# Autodesk Inventor assembly: Assembly1
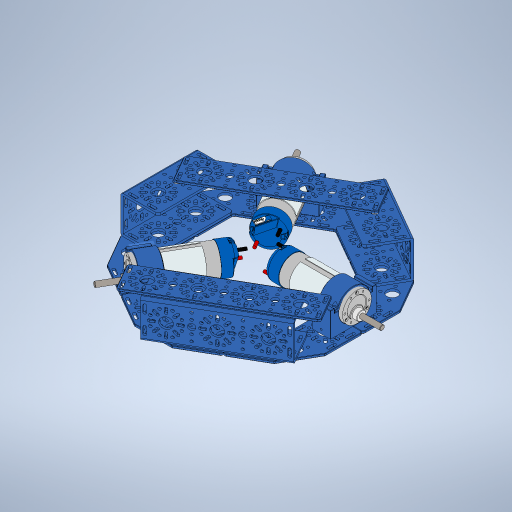
[picture p0: Inventor's stored thumbnail of the model, 512x512]
Saved by Autodesk Inventor 2023 (Build 270158000, 158)
## iProperties
Created: 2022-11-05
Part Number: Assembly1
Document SubType Name: Assembly
Designer: amagw
Author: amagw
## Documents named in this file (9)
- C:\Users\amagw\OneDrive\Документы\Inventor\Assembly1.iam
- C:\Users\amagw\Downloads\76080-120-degree-bracket.ipt
- C:\Users\amagw\Downloads\76017-96mm-u-channel.ipt
- C:\Users\amagw\Downloads\76016-144mm-u-channel.ipt
- C:\Users\amagw\Downloads\76141b-motor-mount-clamp-bottom.ipt
- C:\Users\amagw\Downloads\75001 - Maverick Motor, Spur Gearbox and Encoder.ipt
- C:\Users\amagw\Downloads\76141t-motor-mount-clamp-kit-top.ipt
- C:\Users\amagw\Downloads\76063-192mm-40mm-flat-bracket(1).ipt
- C:\Users\amagw\Downloads\76063-192mm-40mm-flat-bracket(2).ipt
## Components (20 placed, 8 different names)
1. 76063-192mm-40mm-flat-bracket(1):1 — Angle:7, Rotational:14, Rotational:15
2. 76063-192mm-40mm-flat-bracket(2):1 — Angle:8, Rotational:17
3. 76017-96mm-u-channel:2 — Rotational:1, Rotational:2
4. 76016-144mm-u-channel:2 — Rotational:6, Rotational:7, Angle:7, Rotational:14, Rotational:15
5. 76017-96mm-u-channel:1 — Rotational:3, Rotational:4, Rotational:17
6. 76080-120-degree-bracket:1 — Rigid:1, Rotational:6, Rotational:7
7. 76080-120-degree-bracket:2 — Rigid:1, Rigid:2, Rotational:8, Angle:1, Angle:6
8. 76080-120-degree-bracket:3 — Rigid:2, Rigid:3, Rotational:1
9. 76080-120-degree-bracket:4 — Rigid:3, Rigid:4, Rotational:2, Angle:3, Angle:8
10. 76080-120-degree-bracket:5 — Rigid:4, Rigid:5, Rotational:3, Angle:2
11. 76080-120-degree-bracket:6 — Rigid:5, Rotational:4, Angle:4, Angle:5
12. 76141b-motor-mount-clamp-bottom:1 — Angle:4, Angle:5, Rigid:6, Rotational:13, Rotational:16
13. 76141b-motor-mount-clamp-bottom:2 — Angle:2, Angle:3, Rigid:9, Rotational:9, Rotational:10
14. 76141b-motor-mount-clamp-bottom:3 — Rotational:8, Angle:1, Angle:6, Rigid:8, Rotational:11, Rotational:12
15. 75001 - Maverick Motor, Spur Gearbox and Encoder:1 — Rigid:6
16. 75001 - Maverick Motor, Spur Gearbox and Encoder:2 — Rigid:8
17. 75001 - Maverick Motor, Spur Gearbox and Encoder:3 — Rigid:9
18. 76141t-motor-mount-clamp-kit-top:1 — Rotational:11, Rotational:12
19. 76141t-motor-mount-clamp-kit-top:2 — Rotational:13, Rotational:16
20. 76141t-motor-mount-clamp-kit-top:3 — Rotational:9, Rotational:10
## Relationships (32: RevoluteJoint 16, WeldJoint 8, Angle 8)
- Rigid:1 [WeldJoint]: 76080-120-degree-bracket:1 ↔ 76080-120-degree-bracket:2
- Rigid:2 [WeldJoint]: 76080-120-degree-bracket:2 ↔ 76080-120-degree-bracket:3
- Rigid:3 [WeldJoint]: 76080-120-degree-bracket:3 ↔ 76080-120-degree-bracket:4
- Rigid:4 [WeldJoint]: 76080-120-degree-bracket:4 ↔ 76080-120-degree-bracket:5
- Rigid:5 [WeldJoint]: 76080-120-degree-bracket:5 ↔ 76080-120-degree-bracket:6
- Rotational:1 [RevoluteJoint]: 76017-96mm-u-channel:2 ↔ 76080-120-degree-bracket:3
- Rotational:2 [RevoluteJoint]: 76017-96mm-u-channel:2 ↔ 76080-120-degree-bracket:4
- Rotational:3 [RevoluteJoint]: 76017-96mm-u-channel:1 ↔ 76080-120-degree-bracket:5
- Rotational:4 [RevoluteJoint]: 76017-96mm-u-channel:1 ↔ 76080-120-degree-bracket:6
- Rotational:6 [RevoluteJoint]: 76016-144mm-u-channel:2 ↔ 76080-120-degree-bracket:1
- Rotational:7 [RevoluteJoint]: 76016-144mm-u-channel:2 ↔ 76080-120-degree-bracket:1
- Rotational:8 [RevoluteJoint]: 76080-120-degree-bracket:2 ↔ 76141b-motor-mount-clamp-bottom:3
- Angle:1 (0 deg): 76080-120-degree-bracket:2 ↔ 76141b-motor-mount-clamp-bottom:3
- Angle:2 (180 deg): 76080-120-degree-bracket:5 ↔ 76141b-motor-mount-clamp-bottom:2
- Angle:3 (0 deg): 76080-120-degree-bracket:4 ↔ 76141b-motor-mount-clamp-bottom:2
- Angle:4 (180 deg): 76080-120-degree-bracket:6 ↔ 76141b-motor-mount-clamp-bottom:1
- Angle:5 (0 deg): 76080-120-degree-bracket:6 ↔ 76141b-motor-mount-clamp-bottom:1
- Angle:6 (0 deg): 76080-120-degree-bracket:2 ↔ 76141b-motor-mount-clamp-bottom:3
- Rigid:6 [WeldJoint] (-5 mm): 76141b-motor-mount-clamp-bottom:1 ↔ 75001 - Maverick Motor, Spur Gearbox and Encoder:1
- Rigid:8 [WeldJoint] (5 mm): 76141b-motor-mount-clamp-bottom:3 ↔ 75001 - Maverick Motor, Spur Gearbox and Encoder:2
- Rigid:9 [WeldJoint] (-5 mm): 76141b-motor-mount-clamp-bottom:2 ↔ 75001 - Maverick Motor, Spur Gearbox and Encoder:3
- Rotational:9 [RevoluteJoint]: 76141b-motor-mount-clamp-bottom:2 ↔ 76141t-motor-mount-clamp-kit-top:3
- Rotational:10 [RevoluteJoint]: 76141b-motor-mount-clamp-bottom:2 ↔ 76141t-motor-mount-clamp-kit-top:3
- Rotational:11 [RevoluteJoint]: 76141b-motor-mount-clamp-bottom:3 ↔ 76141t-motor-mount-clamp-kit-top:1
- Rotational:12 [RevoluteJoint]: 76141b-motor-mount-clamp-bottom:3 ↔ 76141t-motor-mount-clamp-kit-top:1
- Rotational:13 [RevoluteJoint]: 76141b-motor-mount-clamp-bottom:1 ↔ 76141t-motor-mount-clamp-kit-top:2
- Angle:7 (0 deg): 76063-192mm-40mm-flat-bracket(1):1 ↔ 76016-144mm-u-channel:2
- Rotational:14 [RevoluteJoint]: 76063-192mm-40mm-flat-bracket(1):1 ↔ 76016-144mm-u-channel:2
- Rotational:15 [RevoluteJoint]: 76063-192mm-40mm-flat-bracket(1):1 ↔ 76016-144mm-u-channel:2
- Rotational:16 [RevoluteJoint]: 76141b-motor-mount-clamp-bottom:1 ↔ 76141t-motor-mount-clamp-kit-top:2
- Angle:8 (0 deg): 76063-192mm-40mm-flat-bracket(2):1 ↔ 76080-120-degree-bracket:4
- Rotational:17 [RevoluteJoint]: 76063-192mm-40mm-flat-bracket(2):1 ↔ 76017-96mm-u-channel:1
